# Autodesk Inventor assembly: Assembly2
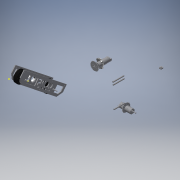
[picture p0: Inventor's stored thumbnail of the model, 180x180]
Saved by Autodesk Inventor 2017 (Build 210142000, 142)
## iProperties
Created: 2017-08-23
Part Number: Assembly2
Document SubType Name: Assembly
Designer: User
Author: User
## Documents named in this file (11)
- C:\Robotics\CAD\2016-17_CAD\DriveTrain\Assembly2.iam
- C:\Robotics\CAD\2016-17_CAD\DriveTrain\drive train standoff.ipt
- C:\Robotics\CAD\2016-17_CAD\DriveTrain\DrainTrainPlate2.0LeftOutside.iam
- C:\Robotics\CAD\2016-17_CAD\DriveTrain\DriveTrainPlate2.0LeftInside.ipt
- C:\Robotics\CAD\COTSParts\Motors\Andymark 2964  NeveRest 40 Motor.ipt
- C:\Robotics\CAD\COTSParts\Tetrix\tetrix-motor-mounts-1.snapshot.1\Tetrex 2pc motor mount.ipt
- C:\Robotics\CAD\COTSParts\Actobotics\615 parts\615114.ipt
- C:\Robotics\CAD\COTSParts\Actobotics\545 parts\545456.ipt
- C:\Robotics\CAD\COTSParts\Actobotics\545 parts\545556.ipt
- C:\Robotics\CAD\COTSParts\Actobotics\634 parts\634080.ipt
- C:\Robotics\CAD\COTSParts\Wheels\4in Wheel Intergreated Hub 8mm Rev2.ipt
## Components (28 placed, 10 different names)
1. drive train standoff:1
2. drive train standoff:2
3. drive train standoff:3
4. DrainTrainPlate2.0LeftOutside:1 [sub-assembly] — Mate:39, Mate:40, Mate:45
5. DriveTrainPlate2.0LeftInside:1 — Mate:37, Mate:38, Mate:41, Mate:42, Mate:43, Mate:44, Mate:46, Mate:47
6. Andymark 2964  NeveRest 40 Motor:1
7. Andymark 2964  NeveRest 40 Motor:2
8. Tetrex 2pc motor mount:1 — Mate:46, Mate:47
9. Tetrex 2pc motor mount:2
10. 615114:1 — Mate:45
11. 615114:2
12. 615114:3
13. 615114:4
14. 545456:1
15. 545456:2
16. 545456:3
17. 545456:4
18. 545556:1
19. 545556:2
20. 545556:3
21. 545556:4
22. 634080:1 — Mate:37, Mate:39, Mate:42
23. 634080:2 — Mate:38, Mate:40, Mate:41
24. 545556:5
25. 545556:6 — Mate:43
26. 4in Wheel Intergreated Hub 8mm Rev2:1
27. 4in Wheel Intergreated Hub 8mm Rev2:2
28. 545556:7 — Mate:44
## Relationships (41: Mate 39, Flush 2)
- [Mate]: 634080:2 ↔ 4in Wheel Intergreated Hub 8mm Rev2:1
- [Mate]: 545456:3 ↔ 4in Wheel Intergreated Hub 8mm Rev2:1
- [Mate]: 545456:3 ↔ 634080:2
- [Mate]: 545456:3 ↔ 545556:2
- [Mate]: 545556:2 ↔ 634080:2
- [Mate]: 615114:1 ↔ 545556:2
- [Mate]: 615114:1 ↔ 634080:2
- [Mate]: 545456:4 ↔ 4in Wheel Intergreated Hub 8mm Rev2:1
- [Mate]: 545456:4 ↔ 634080:2
- [Mate]: 634080:1 ↔ 4in Wheel Intergreated Hub 8mm Rev2:2
- [Mate]: 545456:2 ↔ 4in Wheel Intergreated Hub 8mm Rev2:2
- [Mate]: 545456:2 ↔ 634080:1
- [Mate]: 545456:2 ↔ 545556:1
- [Mate]: 545556:1 ↔ 634080:1
- [Mate]: 615114:3 ↔ 545556:1
- [Mate]: 615114:3 ↔ 634080:1
- [Mate]: 545456:1 ↔ 4in Wheel Intergreated Hub 8mm Rev2:2
- [Mate]: 545456:1 ↔ 634080:1
- [Mate]: 545456:1 ↔ 545556:6
- [Mate]: 634080:1 ↔ 545556:6
- [Mate]: 545456:4 ↔ 545556:7
- [Mate]: 634080:2 ↔ 545556:7
- [Flush]: DrainTrainPlate2.0LeftOutside:1 ↔ DriveTrainPlate2.0LeftInside:1
- [Mate]: Andymark 2964  NeveRest 40 Motor:2 ↔ Tetrex 2pc motor mount:2
- [Mate]: Andymark 2964  NeveRest 40 Motor:2 ↔ 545556:4
- [Mate]: 615114:4 ↔ 545556:4
- [Flush]: 615114:4 ↔ 545556:4
- [Mate]: Andymark 2964  NeveRest 40 Motor:1 ↔ 545556:3
- [Mate]: 615114:2 ↔ 545556:3
- [Mate]: Andymark 2964  NeveRest 40 Motor:1 ↔ 615114:2
- Mate:37: DriveTrainPlate2.0LeftInside:1 ↔ 634080:1
- Mate:38: DriveTrainPlate2.0LeftInside:1 ↔ 634080:2
- Mate:39: DrainTrainPlate2.0LeftOutside:1 ↔ 634080:1
- Mate:40: DrainTrainPlate2.0LeftOutside:1 ↔ 634080:2
- Mate:41: DriveTrainPlate2.0LeftInside:1 ↔ 634080:2
- Mate:42: DriveTrainPlate2.0LeftInside:1 ↔ 634080:1
- Mate:43 (3.175 mm): DriveTrainPlate2.0LeftInside:1 ↔ 545556:6
- Mate:44 (3.175 mm): DriveTrainPlate2.0LeftInside:1 ↔ 545556:7
- Mate:45 (6.35 mm): DrainTrainPlate2.0LeftOutside:1 ↔ 615114:1
- Mate:46: DriveTrainPlate2.0LeftInside:1 ↔ Tetrex 2pc motor mount:1
- Mate:47: DriveTrainPlate2.0LeftInside:1 ↔ Tetrex 2pc motor mount:1
## Named parameters: d35_d36 = 0 mm
